# Autodesk Inventor assembly: flipper_tensioner
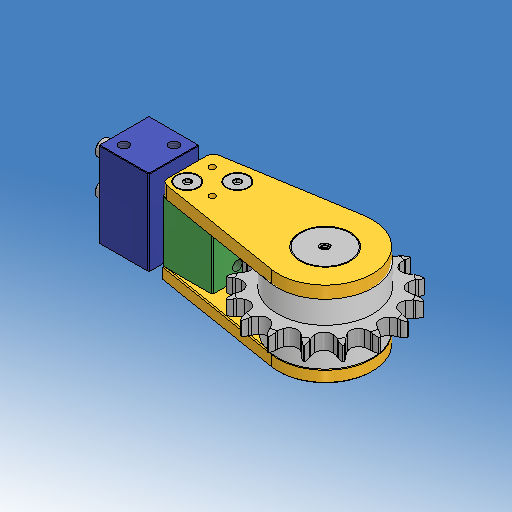
[picture p0: Inventor's stored thumbnail of the model, 512x512]
Saved by Autodesk Inventor 2025 (Build 290162000, 162)
## iProperties
Created: 2023-02-28
Part Number: flipper_tensioner
Document SubType Name: Assembly
Designer: ralph
Author: ralph
## Documents named in this file (10)
- C:\Users\seene\Desktop\Stony Brook\SBRT\RCR_Dexter\Drive\v1\TANK flipper\flipper_tensioner _belt.iam
- C:\Users\seene\Desktop\Stony Brook\SBRT\RCR_Dexter\Drive\v1\TANK flipper\Idler Shaft.ipt
- C:\Users\seene\Desktop\Stony Brook\SBRT\RCR_Dexter\Drive\v1\TANK flipper\tensioner anchor block.ipt
- C:\Users\seene\Desktop\Stony Brook\SBRT\RCR_Dexter\Drive\v1\TANK flipper\tensioner inside plate.ipt
- C:\Users\seene\Desktop\Stony Brook\SBRT\RCR_Dexter\Drive\v1\TANK flipper\tensioner mobile block.ipt
- C:\Users\seene\Desktop\Stony Brook\SBRT\RCR_Dexter\Drive\v1\TANK flipper\tensioner outside plate.ipt
- C:\Users\seene\Desktop\Stony Brook\SBRT\RCR_Dexter\Drive\v1\TANK flipper\91253A245_Black-Oxide Alloy Steel Hex Drive Flat Head Screw v1.ipt
- C:\Users\seene\Desktop\Stony Brook\SBRT\RCR_Dexter\Drive\v1\TANK flipper\90128A229_Zinc-Plated Alloy Steel Socket Head Screw (1) v1.ipt
- C:\Users\seene\Desktop\Stony Brook\SBRT\RCR_Dexter\Drive\v1\TANK flipper\2868T199_High-Load Oil-Embedded 863 Sleeve Bearing (1) v2.ipt
- C:\Users\seene\Desktop\Stony Brook\SBRT\RCR_Dexter\Drive\v1\TANK flipper\Idler Sprocket 16t v12.iam
## Components (13 placed, 9 different names)
1. Idler Shaft:1 — Mate:13, Flush:1, Mate:21, Mate:24
2. tensioner anchor block:1 — Mate:9, Mate:10, Mate:19
3. tensioner inside plate:1 — Mate:1, Mate:2, Mate:3, Mate:4, Mate:5, Mate:14, Flush:3, Mate:15, Flush:4, Mate:25
4. tensioner mobile block:1 — Mate:1, Mate:2, Mate:3, Mate:6, Mate:9, Mate:10, Mate:11, Mate:12, Mate:26
5. tensioner outside plate:1 — Mate:4, Mate:5, Mate:6, Mate:13, Flush:1, Mate:16, Mate:17, Flush:5, Flush:6
6. 91253A245_Black-Oxide Alloy Steel Hex Drive Flat Head Screw v1:2 — Mate:15, Flush:4
7. 91253A245_Black-Oxide Alloy Steel Hex Drive Flat Head Screw v1:3 — Mate:14, Flush:3
8. 91253A245_Black-Oxide Alloy Steel Hex Drive Flat Head Screw v1:4 — Mate:17, Flush:6
9. 91253A245_Black-Oxide Alloy Steel Hex Drive Flat Head Screw v1:5 — Mate:16, Flush:5
10. 90128A229_Zinc-Plated Alloy Steel Socket Head Screw (1) v1:1 — Mate:11, Flush:2, Mate:19
11. 90128A229_Zinc-Plated Alloy Steel Socket Head Screw (1) v1:2 — Mate:12, Flush:2, Mate:26
12. 2868T199_High-Load Oil-Embedded 863 Sleeve Bearing (1) v2:1 — Mate:21
13. Idler Sprocket 16t v12:1 [sub-assembly] — Mate:24, Mate:25
## Relationships (26: Mate 20, Flush 6)
- Mate:1: tensioner inside plate:1 ↔ tensioner mobile block:1
- Mate:2: tensioner inside plate:1 ↔ tensioner mobile block:1
- Mate:3: tensioner inside plate:1 ↔ tensioner mobile block:1
- Mate:4: tensioner inside plate:1 ↔ tensioner outside plate:1
- Mate:5: tensioner inside plate:1 ↔ tensioner outside plate:1
- Mate:6: tensioner mobile block:1 ↔ tensioner outside plate:1
- Mate:9: tensioner anchor block:1 ↔ tensioner mobile block:1
- Mate:10: tensioner anchor block:1 ↔ tensioner mobile block:1
- Mate:11: tensioner mobile block:1 ↔ 90128A229_Zinc-Plated Alloy Steel Socket Head Screw (1) v1:1
- Mate:12: tensioner mobile block:1 ↔ 90128A229_Zinc-Plated Alloy Steel Socket Head Screw (1) v1:2
- Mate:13: Idler Shaft:1 ↔ tensioner outside plate:1
- Flush:1: Idler Shaft:1 ↔ tensioner outside plate:1
- Flush:2: 90128A229_Zinc-Plated Alloy Steel Socket Head Screw (1) v1:1 ↔ 90128A229_Zinc-Plated Alloy Steel Socket Head Screw (1) v1:2
- Mate:14: tensioner inside plate:1 ↔ 91253A245_Black-Oxide Alloy Steel Hex Drive Flat Head Screw v1:3
- Flush:3: tensioner inside plate:1 ↔ 91253A245_Black-Oxide Alloy Steel Hex Drive Flat Head Screw v1:3
- Mate:15: tensioner inside plate:1 ↔ 91253A245_Black-Oxide Alloy Steel Hex Drive Flat Head Screw v1:2
- Flush:4: tensioner inside plate:1 ↔ 91253A245_Black-Oxide Alloy Steel Hex Drive Flat Head Screw v1:2
- Mate:16: tensioner outside plate:1 ↔ 91253A245_Black-Oxide Alloy Steel Hex Drive Flat Head Screw v1:5
- Mate:17: tensioner outside plate:1 ↔ 91253A245_Black-Oxide Alloy Steel Hex Drive Flat Head Screw v1:4
- Flush:5: tensioner outside plate:1 ↔ 91253A245_Black-Oxide Alloy Steel Hex Drive Flat Head Screw v1:5
- Flush:6: tensioner outside plate:1 ↔ 91253A245_Black-Oxide Alloy Steel Hex Drive Flat Head Screw v1:4
- Mate:19: tensioner anchor block:1 ↔ 90128A229_Zinc-Plated Alloy Steel Socket Head Screw (1) v1:1
- Mate:21: Idler Shaft:1 ↔ 2868T199_High-Load Oil-Embedded 863 Sleeve Bearing (1) v2:1
- Mate:24: Idler Shaft:1 ↔ Idler Sprocket 16t v12:1
- Mate:25: tensioner inside plate:1 ↔ Idler Sprocket 16t v12:1
- Mate:26 (-12.7 mm): tensioner mobile block:1 ↔ 90128A229_Zinc-Plated Alloy Steel Socket Head Screw (1) v1:2
